# Autodesk Inventor assembly: Intel_RealSense_Depth_Camera_D435
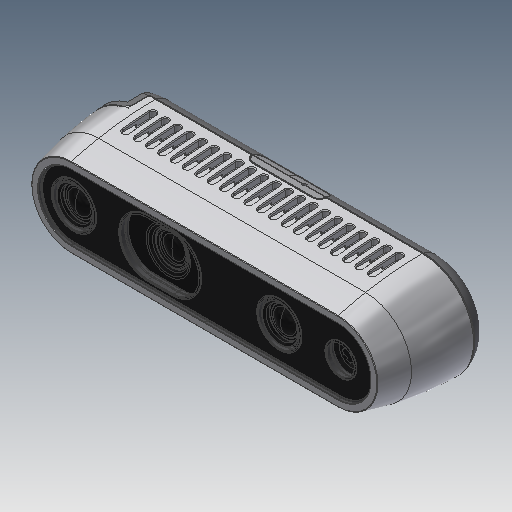
[picture p0: Inventor's stored thumbnail of the model, 512x512]
Saved by Autodesk Inventor 2019.4 (Build 234330000, 330)
## iProperties
Created: 2017-10-02
Part Number: Intel_RealSense_Depth_Camera_D435
Material: 一般
Document SubType Name: Assembly
Designer: y6tada
Author: y6tada
Revision Number: 1LAST_VERSION
## Documents named in this file (10)
- C:\GrabCAD\Yunit 8\Libs\Intel Realsense D435\Intel\Intel_RealSense_Depth_Camera_D435.iam
- C:\GrabCAD\Yunit 8\Libs\Intel Realsense D435\Intel\FRONT_COVER_ALUMINUM_AWG_W_RGB_.ipt
- C:\GrabCAD\Yunit 8\Libs\Intel Realsense D435\Intel\LENS_COVER_SUBASSY_AWG_W_RGB_AS_ASM.iam
- C:\GrabCAD\Yunit 8\Libs\Intel Realsense D435\Intel\FOAM_ISOLATION_CARRIER_AWG_RGB__ASM.iam
- C:\GrabCAD\Yunit 8\Libs\Intel Realsense D435\Intel\CAMERA_MOD_DS5_AWG_ASM_46_ASM.iam
- C:\GrabCAD\Yunit 8\Libs\Intel Realsense D435\Intel\DS5_RGB_MODULE_ASM_13_ASM.iam
- C:\GrabCAD\Yunit 8\Libs\Intel Realsense D435\Intel\HEATSINK_AWG_W_RGB_24.ipt
- C:\GrabCAD\Yunit 8\Libs\Intel Realsense D435\Intel\REAR_COVER_SUBASSY_AWG_W_RGB_AS_ASM.iam
- C:\GrabCAD\Yunit 8\Libs\Intel Realsense D435\Intel\AUX_COVER_SUBASSY_AWG_W_RGB_ASM_ASM.iam
- C:\Users\y6tada\Documents\Inventor\Content Center Files\R2019\ja-JP\ISO 7046-1 H(1)\ISO 7046-1 - M2 x 5 - 4.8 - H - ISO.ipt
## Components (10 placed, 9 different names)
1. 165 [sub-assembly] — メイト:1, メイト:2, フラッシュ:1
2. 123
3. 128 [sub-assembly]
4. 133 [sub-assembly]
5. 141 [sub-assembly]
6. 148 [sub-assembly]
7. 149
8. 171 [sub-assembly]
9. ISO 7046-1 H M2 x 5 - 4.8 - H:1 — メイト:1
10. ISO 7046-1 H M2 x 5 - 4.8 - H:2 — メイト:2
## Relationships (3: Mate 2, Flush 1)
- メイト:1 [Mate]: 165 ↔ ISO 7046-1 H M2 x 5 - 4.8 - H:1
- メイト:2 [Mate]: 165 ↔ ISO 7046-1 H M2 x 5 - 4.8 - H:2
- フラッシュ:1 [Flush] (1.58 mm): 165
